# Autodesk Inventor assembly: Updated
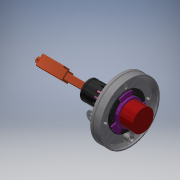
[picture p0: Inventor's stored thumbnail of the model, 180x180]
Saved by Autodesk Inventor 2017 (Build 210142000, 142)
## iProperties
Created: 2017-03-13
Part Number: Updated
Document SubType Name: Assembly
Designer: Joseph
Author: Joseph
## Documents named in this file (14)
- D:\Joseph\Documents\School\College\Clubs\Balloon\2017 Design\Updated.iam
- D:\Joseph\Documents\School\College\Clubs\Balloon\2017 Design\Disc.ipt
- D:\Joseph\Documents\School\College\Clubs\Balloon\2017 Design\LargeO-Ring.ipt
- D:\Joseph\Documents\School\College\Clubs\Balloon\2017 Design\ActuatorCap.ipt
- D:\Joseph\Documents\School\College\Clubs\Balloon\2017 Design\ActuatorRetracted.ipt
- D:\Joseph\Documents\School\College\Clubs\Balloon\2017 Design\Plug.ipt
- D:\Joseph\Documents\School\College\Clubs\Balloon\2017 Design\ValveStem.ipt
- D:\Joseph\Documents\School\College\Clubs\Balloon\2017 Design\ReciprocatingO-Ring.ipt
- D:\Joseph\Documents\School\College\Clubs\Balloon\2017 Design\FillPort.ipt
- D:\Joseph\Documents\School\College\Clubs\Balloon\2017 Design\EyeBolt.ipt
- D:\Joseph\Documents\School\College\Clubs\Balloon\2017 Design\Fan.ipt
- D:\Joseph\Documents\School\College\Clubs\Balloon\2017 Design\FanMount.ipt
- D:\Joseph\Documents\School\College\Clubs\Balloon\2017 Design\FillPlug.ipt
- D:\Joseph\Documents\School\College\Clubs\Balloon\2017 Design\FillPortUpdated.ipt
## Components (14 placed, 13 different names)
1. Disc:1 — Rigid:1, Rigid:4, Rotational:3, Rotational:4, Rigid:11, Rotational:5
2. LargeO-Ring:1 — Rigid:1
3. ActuatorCap:1 — Rigid:12, Rigid:13
4. ActuatorRetracted:1 — Rigid:12
5. Plug:1 — Rigid:5, Cylindrical:1, Rigid:13
6. ValveStem:1 — Rigid:4, Cylindrical:1, Rigid:9
7. ReciprocatingO-Ring:1 — Rigid:5
8. FillPort:1
9. EyeBolt:1 — Rotational:3
10. EyeBolt:2 — Rotational:4
11. Fan:1 — Rigid:9, Rigid:10
12. FanMount:1 — Rigid:10
13. FillPlug:1 — Rigid:11
14. FillPortUpdated:1 — Rotational:5
## Relationships (12: WeldJoint 8, RevoluteJoint 3, CylindricalJoint 1)
- Rigid:1 [WeldJoint] (1.1906 mm): Disc:1 ↔ LargeO-Ring:1
- Rigid:4 [WeldJoint]: Disc:1 ↔ ValveStem:1
- Rigid:5 [WeldJoint]: Plug:1 ↔ ReciprocatingO-Ring:1
- Cylindrical:1: Plug:1 ↔ ValveStem:1
- Rotational:3 [RevoluteJoint] (-5.08 mm): Disc:1 ↔ EyeBolt:1
- Rotational:4 [RevoluteJoint] (-5.08 mm): Disc:1 ↔ EyeBolt:2
- Rigid:9 [WeldJoint]: ValveStem:1 ↔ Fan:1
- Rigid:10 [WeldJoint]: Fan:1 ↔ FanMount:1
- Rigid:11 [WeldJoint]: Disc:1 ↔ FillPlug:1
- Rotational:5 [RevoluteJoint]: Disc:1 ↔ FillPortUpdated:1
- Rigid:12 [WeldJoint]: ActuatorCap:1 ↔ ActuatorRetracted:1
- Rigid:13 [WeldJoint]: ActuatorCap:1 ↔ Plug:1
